# Autodesk Inventor assembly: 新型３クランクアセンブリ_MIR
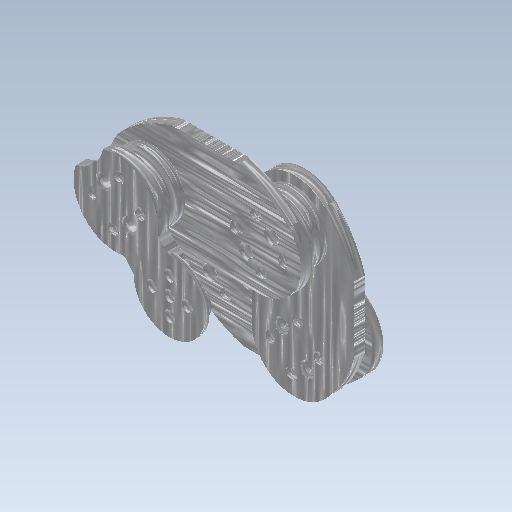
[picture p0: Inventor's stored thumbnail of the model, 512x512]
Saved by Autodesk Inventor 2020 (Build 240168000, 168)
## iProperties
Created: 2019-04-15
Part Number: 新型３クランクアセンブリ_MIR
Material: 一般
Document SubType Name: Assembly
Designer: tanjihayato
Mass: 22.1475 g
Surface Area: 127.97 cm^2
Volume: 7.88167 cm^3
Density: 2.81 g/cm^3
Author: tanjihayato
## Documents named in this file (5)
- \\Mac\Home\Documents\Inventor\2019お遊び機体\新型３クランクアセンブリ_MIR.iam
- \\Mac\Home\Documents\Inventor\2019お遊び機体\新型３クランク_MIR.ipt
- \\Mac\Home\Documents\Inventor\2019お遊び機体\新型３脚カム.ipt
- \\Mac\Home\Documents\Inventor\2019お遊び機体\新型３クランク根本_MIR.ipt
- \\Mac\Home\Documents\Inventor\2019お遊び機体\新型３涙_MIR.ipt
## Components (9 placed, 4 different names)
1. 新型３クランク_MIR:1 — メイト:1, 挿入:1, メイト:7, 挿入:7
2. 新型３クランク_MIR:2 — メイト:2, 挿入:2, メイト:6, 挿入:6
3. 新型３クランク_MIR:3 — メイト:3, 挿入:3, メイト:5, 挿入:5
4. 新型３脚カム:1 — メイト:1, 挿入:1, メイト:8, 挿入:8
5. 新型３脚カム:2 — メイト:7, 挿入:7, メイト:2, 挿入:2
6. 新型３脚カム:3 — メイト:6, 挿入:6, メイト:3, 挿入:3
7. 新型３脚カム:4 — メイト:5, 挿入:5, メイト:4, 挿入:4
8. 新型３クランク根本_MIR:1 — メイト:4, 挿入:4
9. 新型３涙_MIR:1 — メイト:8, 挿入:8
## Relationships (16: Mate 8, Insert 8)
- メイト:1 [Mate]: 新型３クランク_MIR:1 ↔ 新型３脚カム:1
- 挿入:1 [Insert]: 新型３クランク_MIR:1 ↔ 新型３脚カム:1
- メイト:7 [Mate]: 新型３クランク_MIR:1 ↔ 新型３脚カム:2
- 挿入:7 [Insert]: 新型３クランク_MIR:1 ↔ 新型３脚カム:2
- メイト:2 [Mate]: 新型３クランク_MIR:2 ↔ 新型３脚カム:2
- 挿入:2 [Insert]: 新型３クランク_MIR:2 ↔ 新型３脚カム:2
- メイト:6 [Mate]: 新型３クランク_MIR:2 ↔ 新型３脚カム:3
- 挿入:6 [Insert]: 新型３クランク_MIR:2 ↔ 新型３脚カム:3
- メイト:3 [Mate]: 新型３クランク_MIR:3 ↔ 新型３脚カム:3
- 挿入:3 [Insert]: 新型３クランク_MIR:3 ↔ 新型３脚カム:3
- メイト:5 [Mate]: 新型３クランク_MIR:3 ↔ 新型３脚カム:4
- 挿入:5 [Insert]: 新型３クランク_MIR:3 ↔ 新型３脚カム:4
- メイト:4 [Mate]: 新型３脚カム:4 ↔ 新型３クランク根本_MIR:1
- 挿入:4 [Insert]: 新型３脚カム:4 ↔ 新型３クランク根本_MIR:1
- メイト:8 [Mate]: 新型３脚カム:1 ↔ 新型３涙_MIR:1
- 挿入:8 [Insert]: 新型３脚カム:1 ↔ 新型３涙_MIR:1
